# Autodesk Inventor assembly: right pneumatics board
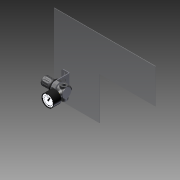
[picture p0: Inventor's stored thumbnail of the model, 180x180]
Saved by Autodesk Inventor 2014 (Build 180170000, 170)
## iProperties
Created: 2014-01-20
Part Number: right pneumatics board
Document SubType Name: Assembly
Designer: Arpan
Author: Arpan
## Documents named in this file (4)
- C:\Users\Andrew Toennies\Documents\GitHub\2014buildCAD\pneumatics board\right pneumatics board.iam
- C:\Users\Andrew Toennies\Documents\GitHub\2014buildCAD\pneumatics board\pneumatics board 1.ipt
- C:\Users\Andrew Toennies\Documents\GitHub\2014buildCAD\pneumatics board\pneumatics thing 2.iam
- C:\Users\Andrew Toennies\Documents\GitHub\2014buildCAD\big air tank\Pneumatics_Clippard_AVT-32-32.iam
## Components (3 placed, 3 different names)
1. pneumatics board 1:1 — Mate:1, Flush:1, Flush:2, Tangent:1, Flush:3
2. pneumatics thing 2:1 [sub-assembly] — Mate:1, Flush:1, Flush:2
3. Pneumatics_Clippard_AVT-32-32:1 [sub-assembly] — Tangent:1, Flush:3
## Relationships (5: Flush 3, Mate 1, Tangent 1)
- Mate:1: pneumatics board 1:1 ↔ pneumatics thing 2:1
- Flush:1 (57.15 mm): pneumatics board 1:1 ↔ pneumatics thing 2:1
- Flush:2 (63.5 mm): pneumatics board 1:1 ↔ pneumatics thing 2:1
- Tangent:1: pneumatics board 1:1 ↔ Pneumatics_Clippard_AVT-32-32:1
- Flush:3: pneumatics board 1:1 ↔ Pneumatics_Clippard_AVT-32-32:1
